# Autodesk Inventor assembly: Сборка крышка
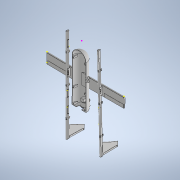
[picture p0: Inventor's stored thumbnail of the model, 180x180]
Saved by Autodesk Inventor 2022.1 (Build 261234000, 234)
## iProperties
Created: 2021-12-25
Part Number: Сборка крышка
Document SubType Name: Assembly
Designer: Grigori
Author: Grigori
## Documents named in this file (19)
- C:\Users\Grigo\Desktop\Дрон\Сборка\Сборка крышка.iam
- C:\Users\Grigo\Desktop\Дрон\Сборка\Корпус1.ipt
- C:\Users\Grigo\Desktop\Дрон\Сборка\Impeller.ipt
- C:\Users\Grigo\Desktop\Дрон\Сборка\Крышка на мотор.ipt
- C:\Users\Grigo\Desktop\Дрон\Сборка\Держатель крыла.ipt
- C:\Users\Grigo\Desktop\Дрон\Сборка\полукрыло.ipt
- C:\Users\Grigo\Desktop\Дрон\Сборка\Продольный фюзеляж.ipt
- C:\Users\Grigo\Desktop\Дрон\Сборка\2207 motor.ipt
- C:\Users\Grigo\Desktop\Дрон\Сборка\esc 80A.ipt
- C:\Users\Grigo\Desktop\Дрон\Сборка\Крышка на ESC.ipt
- C:\Users\Grigo\Desktop\Дрон\Сборка\полукрыло_MIR.ipt
- C:\Users\Grigo\Desktop\Дрон\Сборка\Продольный фюзеляж_MIR.ipt
- C:\Users\Grigo\Desktop\Дрон\Сборка\2207 motor_MIR.ipt
- C:\Users\Grigo\Desktop\Дрон\Сборка\Крышка на ESC_MIR.ipt
- C:\Users\Grigo\Desktop\Дрон\Сборка\esc 80A_MIR.ipt
- C:\Users\Grigo\Documents\Inventor\Content Center Files\R2022\ru-RU\AS 1427(01)\AS 1427 - M3 x 8(3).ipt
- C:\Users\Grigo\Documents\Inventor\Content Center Files\R2022\ru-RU\Rivet JB_T 10582-2006\Rivet JB_T 10582-2006-10 X 25.ipt
- C:\Users\Grigo\Documents\Inventor\Content Center Files\R2022\ru-RU\AS 1427(05)\AS 1427 - M2,5 x 10(5) II.ipt
- C:\Users\Grigo\Documents\Inventor\Content Center Files\R2022\ru-RU\AS 1427(01)\AS 1427 - M3 x 5(3).ipt
## Components (85 placed, 18 different names)
1. Корпус1:1 — С поворотом:1, Совмещение:2, С поворотом:3, С поворотом:4, Жесткий:1, Совмещение:5, Совмещение:25, Совмещение:26, Совмещение:27, Совмещение:28, Совмещение:45
2. Impeller:1 — С поворотом:1, С поворотом:2, Совмещение:45
3. Крышка на мотор:1 — С поворотом:2, Совмещение:2, С поворотом:3, Совмещение:46, Совмещение:47, Совмещение:48, Совмещение:49
4. Держатель крыла:1 — Жесткий:1, Совмещение:3
5. Держатель крыла:2 — С поворотом:4, Совмещение:4
6. полукрыло:1 — Совмещение:3, Совмещение:4, Совмещение:5, Совмещение:6, Совмещение:7, Совмещение:50, Совмещение:51, Совмещение:52
7. Продольный фюзеляж:1 — Совмещение:6, Совмещение:7, Совмещение:8, Совмещение:9, Совмещение:10, Совмещение:11, Совмещение:12, Совмещение:13, Совмещение:14, Совмещение:15, Совмещение:16, Совмещение:17, Совмещение:18, Совмещение:19, Совмещение:20, Совмещение:21, Совмещение:22, Совмещение:23, Совмещение:24, С поворотом:5, С поворотом:6, С поворотом:7, С поворотом:8, С поворотом:9, С поворотом:10, С поворотом:11, С поворотом:12, С поворотом:13, С поворотом:14, С поворотом:15, С поворотом:16
8. 2207 motor:1 — Совмещение:8, Совмещение:11
9. 2207 motor:2 — Совмещение:9, Совмещение:12
10. 2207 motor:3 — Совмещение:10, Совмещение:13
11. esc 80A:1 — Совмещение:14
12. esc 80A:2 — Совмещение:15
13. esc 80A:3 — Совмещение:16
14. Крышка на ESC:1 — Совмещение:22, Совмещение:23, Совмещение:24, С поворотом:37, С поворотом:38, С поворотом:39, С поворотом:40
15. Крышка на ESC:2 — Совмещение:17, Совмещение:18, С поворотом:33, С поворотом:34, С поворотом:35, С поворотом:36
16. Крышка на ESC:3 — Совмещение:19, Совмещение:20, Совмещение:21, С поворотом:29, С поворотом:30, С поворотом:31, С поворотом:32
17. полукрыло_MIR:1 — Совмещение:29, Совмещение:30, Совмещение:53, Совмещение:54, Совмещение:55
18. Продольный фюзеляж_MIR:1 — Совмещение:29, Совмещение:30, Совмещение:31, Совмещение:32, Совмещение:33, Совмещение:34, Совмещение:35, Совмещение:36, Совмещение:37, Совмещение:38, Совмещение:39, Совмещение:40, Совмещение:41, Совмещение:42, Совмещение:43, Совмещение:44, С поворотом:17, С поворотом:18, С поворотом:19, С поворотом:20, С поворотом:21, С поворотом:22, С поворотом:23, С поворотом:24, С поворотом:25, С поворотом:26, С поворотом:27, С поворотом:28
19. 2207 motor_MIR:1 — Совмещение:31, Совмещение:32
20. 2207 motor_MIR:2 — Совмещение:33, Совмещение:34
21. 2207 motor_MIR:3 — Совмещение:35, Совмещение:36
22. Крышка на ESC_MIR:1 — Совмещение:37, Совмещение:38, Совмещение:39, С поворотом:41, С поворотом:42, С поворотом:43, С поворотом:44
23. Крышка на ESC_MIR:2 — Совмещение:40, Совмещение:41, С поворотом:45, С поворотом:46, С поворотом:47, С поворотом:48
24. Крышка на ESC_MIR:3 — Совмещение:42, Совмещение:43, Совмещение:44, С поворотом:49, С поворотом:50, С поворотом:51, С поворотом:52
25. esc 80A_MIR:1
26. esc 80A_MIR:2
27. esc 80A_MIR:3
28. AS 1427 - метрическая M3 x 8:1 — Совмещение:46
29. AS 1427 - метрическая M3 x 8:2 — Совмещение:48
30. AS 1427 - метрическая M3 x 8:3 — Совмещение:47
31. AS 1427 - метрическая M3 x 8:4 — Совмещение:49
32. Rivet JB/T 10582-2006 10 X 25:1 — Совмещение:52
33. Rivet JB/T 10582-2006 10 X 25:2 — Совмещение:51
34. Rivet JB/T 10582-2006 10 X 25:3 — Совмещение:50
35. Rivet JB/T 10582-2006 10 X 25:4 — Совмещение:55
36. Rivet JB/T 10582-2006 10 X 25:5 — Совмещение:54
37. Rivet JB/T 10582-2006 10 X 25:6 — Совмещение:53
38. AS 1427 H - метрическая M2,5 x 10:1 — С поворотом:5
39. AS 1427 H - метрическая M2,5 x 10:2 — С поворотом:8
40. AS 1427 H - метрическая M2,5 x 10:3 — С поворотом:7
41. AS 1427 H - метрическая M2,5 x 10:4 — С поворотом:6
42. AS 1427 H - метрическая M2,5 x 10:5 — С поворотом:9
43. AS 1427 H - метрическая M2,5 x 10:6 — С поворотом:10
44. AS 1427 H - метрическая M2,5 x 10:7 — С поворотом:11
45. AS 1427 H - метрическая M2,5 x 10:8 — С поворотом:12
46. AS 1427 H - метрическая M2,5 x 10:9 — С поворотом:16
47. AS 1427 H - метрическая M2,5 x 10:10 — С поворотом:15
48. AS 1427 H - метрическая M2,5 x 10:11 — С поворотом:13
49. AS 1427 H - метрическая M2,5 x 10:12 — С поворотом:14
50. AS 1427 H - метрическая M2,5 x 10:13 — С поворотом:19
51. AS 1427 H - метрическая M2,5 x 10:14 — С поворотом:17
52. AS 1427 H - метрическая M2,5 x 10:15 — С поворотом:18
53. AS 1427 H - метрическая M2,5 x 10:16 — С поворотом:20
54. AS 1427 H - метрическая M2,5 x 10:17 — С поворотом:22
55. AS 1427 H - метрическая M2,5 x 10:18 — С поворотом:21
56. AS 1427 H - метрическая M2,5 x 10:19 — С поворотом:23
57. AS 1427 H - метрическая M2,5 x 10:20 — С поворотом:24
58. AS 1427 H - метрическая M2,5 x 10:21 — С поворотом:27
59. AS 1427 H - метрическая M2,5 x 10:22 — С поворотом:25
60. AS 1427 H - метрическая M2,5 x 10:23 — С поворотом:26
61. AS 1427 H - метрическая M2,5 x 10:24 — С поворотом:28
62. AS 1427 - метрическая M3 x 5:1 — С поворотом:29
63. AS 1427 - метрическая M3 x 5:2 — С поворотом:30
64. AS 1427 - метрическая M3 x 5:3 — С поворотом:31
65. AS 1427 - метрическая M3 x 5:4 — С поворотом:32
66. AS 1427 - метрическая M3 x 5:5 — С поворотом:34
67. AS 1427 - метрическая M3 x 5:6 — С поворотом:33
68. AS 1427 - метрическая M3 x 5:7 — С поворотом:35
69. AS 1427 - метрическая M3 x 5:8 — С поворотом:36
70. AS 1427 - метрическая M3 x 5:9 — С поворотом:38
71. AS 1427 - метрическая M3 x 5:10 — С поворотом:37
72. AS 1427 - метрическая M3 x 5:11 — С поворотом:39
73. AS 1427 - метрическая M3 x 5:12 — С поворотом:40
74. AS 1427 - метрическая M3 x 5:13 — С поворотом:41
75. AS 1427 - метрическая M3 x 5:14 — С поворотом:42
76. AS 1427 - метрическая M3 x 5:15 — С поворотом:44
77. AS 1427 - метрическая M3 x 5:16 — С поворотом:43
78. AS 1427 - метрическая M3 x 5:17 — С поворотом:45
79. AS 1427 - метрическая M3 x 5:18 — С поворотом:46
80. AS 1427 - метрическая M3 x 5:19 — С поворотом:48
81. AS 1427 - метрическая M3 x 5:20 — С поворотом:47
82. AS 1427 - метрическая M3 x 5:21 — С поворотом:49
83. AS 1427 - метрическая M3 x 5:22 — С поворотом:50
84. AS 1427 - метрическая M3 x 5:23 — С поворотом:52
85. AS 1427 - метрическая M3 x 5:24 — С поворотом:51
## Relationships (108: Mate 54, RevoluteJoint 52, WeldJoint 1, Symmetry 1)
- С поворотом:1 [RevoluteJoint]: Корпус1:1 ↔ Impeller:1
- С поворотом:2 [RevoluteJoint]: Impeller:1 ↔ Крышка на мотор:1
- Совмещение:2 [Mate]: Корпус1:1 ↔ Крышка на мотор:1
- С поворотом:3 [RevoluteJoint]: Корпус1:1 ↔ Крышка на мотор:1
- С поворотом:4 [RevoluteJoint]: Корпус1:1 ↔ Держатель крыла:2
- Жесткий:1 [WeldJoint]: Корпус1:1 ↔ Держатель крыла:1
- Совмещение:3 [Mate]: Держатель крыла:1 ↔ полукрыло:1
- Совмещение:4 [Mate]: Держатель крыла:2 ↔ полукрыло:1
- Совмещение:5 [Mate]: Корпус1:1 ↔ полукрыло:1
- Совмещение:6 [Mate]: полукрыло:1 ↔ Продольный фюзеляж:1
- Совмещение:7 [Mate]: полукрыло:1 ↔ Продольный фюзеляж:1
- Совмещение:8 [Mate]: Продольный фюзеляж:1 ↔ 2207 motor:1
- Совмещение:9 [Mate]: Продольный фюзеляж:1 ↔ 2207 motor:2
- Совмещение:10 [Mate]: Продольный фюзеляж:1 ↔ 2207 motor:3
- Совмещение:11 [Mate]: Продольный фюзеляж:1 ↔ 2207 motor:1
- Совмещение:12 [Mate]: Продольный фюзеляж:1 ↔ 2207 motor:2
- Совмещение:13 [Mate]: Продольный фюзеляж:1 ↔ 2207 motor:3
- Совмещение:14 [Mate]: Продольный фюзеляж:1 ↔ esc 80A:1
- Совмещение:15 [Mate]: Продольный фюзеляж:1 ↔ esc 80A:2
- Совмещение:16 [Mate]: Продольный фюзеляж:1 ↔ esc 80A:3
- Совмещение:17 [Mate]: Продольный фюзеляж:1 ↔ Крышка на ESC:2
- Совмещение:18 [Mate]: Продольный фюзеляж:1 ↔ Крышка на ESC:2
- Совмещение:19 [Mate]: Продольный фюзеляж:1 ↔ Крышка на ESC:3
- Совмещение:20 [Mate]: Продольный фюзеляж:1 ↔ Крышка на ESC:3
- Совмещение:21 [Mate]: Продольный фюзеляж:1 ↔ Крышка на ESC:3
- Совмещение:22 [Mate]: Продольный фюзеляж:1 ↔ Крышка на ESC:1
- Совмещение:23 [Mate]: Продольный фюзеляж:1 ↔ Крышка на ESC:1
- Совмещение:24 [Mate]: Продольный фюзеляж:1 ↔ Крышка на ESC:1
- Совмещение:25 [Mate]: Корпус1:1
- Совмещение:26 [Mate]: Корпус1:1
- Совмещение:27 [Mate]: Корпус1:1
- Совмещение:28 [Mate]: Корпус1:1
- Симметрия:1 [Symmetry]
- Совмещение:29 [Mate]: полукрыло_MIR:1 ↔ Продольный фюзеляж_MIR:1
- Совмещение:30 [Mate]: полукрыло_MIR:1 ↔ Продольный фюзеляж_MIR:1
- Совмещение:31 [Mate]: Продольный фюзеляж_MIR:1 ↔ 2207 motor_MIR:1
- Совмещение:32 [Mate]: Продольный фюзеляж_MIR:1 ↔ 2207 motor_MIR:1
- Совмещение:33 [Mate]: Продольный фюзеляж_MIR:1 ↔ 2207 motor_MIR:2
- Совмещение:34 [Mate]: Продольный фюзеляж_MIR:1 ↔ 2207 motor_MIR:2
- Совмещение:35 [Mate]: Продольный фюзеляж_MIR:1 ↔ 2207 motor_MIR:3
- Совмещение:36 [Mate]: Продольный фюзеляж_MIR:1 ↔ 2207 motor_MIR:3
- Совмещение:37 [Mate]: Продольный фюзеляж_MIR:1 ↔ Крышка на ESC_MIR:1
- Совмещение:38 [Mate]: Продольный фюзеляж_MIR:1 ↔ Крышка на ESC_MIR:1
- Совмещение:39 [Mate]: Продольный фюзеляж_MIR:1 ↔ Крышка на ESC_MIR:1
- Совмещение:40 [Mate]: Продольный фюзеляж_MIR:1 ↔ Крышка на ESC_MIR:2
- Совмещение:41 [Mate]: Продольный фюзеляж_MIR:1 ↔ Крышка на ESC_MIR:2
- Совмещение:42 [Mate]: Продольный фюзеляж_MIR:1 ↔ Крышка на ESC_MIR:3
- Совмещение:43 [Mate]: Продольный фюзеляж_MIR:1 ↔ Крышка на ESC_MIR:3
- Совмещение:44 [Mate]: Продольный фюзеляж_MIR:1 ↔ Крышка на ESC_MIR:3
- Совмещение:45 [Mate]: Корпус1:1 ↔ Impeller:1
- Совмещение:46 [Mate]: Крышка на мотор:1 ↔ AS 1427 - метрическая M3 x 8:1
- Совмещение:47 [Mate]: Крышка на мотор:1 ↔ AS 1427 - метрическая M3 x 8:3
- Совмещение:48 [Mate]: Крышка на мотор:1 ↔ AS 1427 - метрическая M3 x 8:2
- Совмещение:49 [Mate]: Крышка на мотор:1 ↔ AS 1427 - метрическая M3 x 8:4
- Совмещение:50 [Mate]: полукрыло:1 ↔ Rivet JB/T 10582-2006 10 X 25:3
- Совмещение:51 [Mate]: полукрыло:1 ↔ Rivet JB/T 10582-2006 10 X 25:2
- Совмещение:52 [Mate]: полукрыло:1 ↔ Rivet JB/T 10582-2006 10 X 25:1
- Совмещение:53 [Mate]: полукрыло_MIR:1 ↔ Rivet JB/T 10582-2006 10 X 25:6
- Совмещение:54 [Mate]: полукрыло_MIR:1 ↔ Rivet JB/T 10582-2006 10 X 25:5
- Совмещение:55 [Mate]: полукрыло_MIR:1 ↔ Rivet JB/T 10582-2006 10 X 25:4
- С поворотом:5 [RevoluteJoint]: Продольный фюзеляж:1 ↔ AS 1427 H - метрическая M2,5 x 10:1
- С поворотом:6 [RevoluteJoint]: Продольный фюзеляж:1 ↔ AS 1427 H - метрическая M2,5 x 10:4
- С поворотом:7 [RevoluteJoint]: Продольный фюзеляж:1 ↔ AS 1427 H - метрическая M2,5 x 10:3
- С поворотом:8 [RevoluteJoint]: Продольный фюзеляж:1 ↔ AS 1427 H - метрическая M2,5 x 10:2
- С поворотом:9 [RevoluteJoint]: Продольный фюзеляж:1 ↔ AS 1427 H - метрическая M2,5 x 10:5
- С поворотом:10 [RevoluteJoint]: Продольный фюзеляж:1 ↔ AS 1427 H - метрическая M2,5 x 10:6
- С поворотом:11 [RevoluteJoint]: Продольный фюзеляж:1 ↔ AS 1427 H - метрическая M2,5 x 10:7
- С поворотом:12 [RevoluteJoint]: Продольный фюзеляж:1 ↔ AS 1427 H - метрическая M2,5 x 10:8
- С поворотом:13 [RevoluteJoint]: Продольный фюзеляж:1 ↔ AS 1427 H - метрическая M2,5 x 10:11
- С поворотом:14 [RevoluteJoint]: Продольный фюзеляж:1 ↔ AS 1427 H - метрическая M2,5 x 10:12
- С поворотом:15 [RevoluteJoint]: Продольный фюзеляж:1 ↔ AS 1427 H - метрическая M2,5 x 10:10
- С поворотом:16 [RevoluteJoint]: Продольный фюзеляж:1 ↔ AS 1427 H - метрическая M2,5 x 10:9
- С поворотом:17 [RevoluteJoint]: Продольный фюзеляж_MIR:1 ↔ AS 1427 H - метрическая M2,5 x 10:14
- С поворотом:18 [RevoluteJoint]: Продольный фюзеляж_MIR:1 ↔ AS 1427 H - метрическая M2,5 x 10:15
- С поворотом:19 [RevoluteJoint]: Продольный фюзеляж_MIR:1 ↔ AS 1427 H - метрическая M2,5 x 10:13
- С поворотом:20 [RevoluteJoint]: Продольный фюзеляж_MIR:1 ↔ AS 1427 H - метрическая M2,5 x 10:16
- С поворотом:21 [RevoluteJoint]: Продольный фюзеляж_MIR:1 ↔ AS 1427 H - метрическая M2,5 x 10:18
- С поворотом:22 [RevoluteJoint]: Продольный фюзеляж_MIR:1 ↔ AS 1427 H - метрическая M2,5 x 10:17
- С поворотом:23 [RevoluteJoint]: Продольный фюзеляж_MIR:1 ↔ AS 1427 H - метрическая M2,5 x 10:19
- С поворотом:24 [RevoluteJoint]: Продольный фюзеляж_MIR:1 ↔ AS 1427 H - метрическая M2,5 x 10:20
- С поворотом:25 [RevoluteJoint]: Продольный фюзеляж_MIR:1 ↔ AS 1427 H - метрическая M2,5 x 10:22
- С поворотом:26 [RevoluteJoint]: Продольный фюзеляж_MIR:1 ↔ AS 1427 H - метрическая M2,5 x 10:23
- С поворотом:27 [RevoluteJoint]: Продольный фюзеляж_MIR:1 ↔ AS 1427 H - метрическая M2,5 x 10:21
- С поворотом:28 [RevoluteJoint]: Продольный фюзеляж_MIR:1 ↔ AS 1427 H - метрическая M2,5 x 10:24
- С поворотом:29 [RevoluteJoint]: Крышка на ESC:3 ↔ AS 1427 - метрическая M3 x 5:1
- С поворотом:30 [RevoluteJoint]: Крышка на ESC:3 ↔ AS 1427 - метрическая M3 x 5:2
- С поворотом:31 [RevoluteJoint]: Крышка на ESC:3 ↔ AS 1427 - метрическая M3 x 5:3
- С поворотом:32 [RevoluteJoint]: Крышка на ESC:3 ↔ AS 1427 - метрическая M3 x 5:4
- С поворотом:33 [RevoluteJoint]: Крышка на ESC:2 ↔ AS 1427 - метрическая M3 x 5:6
- С поворотом:34 [RevoluteJoint]: Крышка на ESC:2 ↔ AS 1427 - метрическая M3 x 5:5
- С поворотом:35 [RevoluteJoint]: Крышка на ESC:2 ↔ AS 1427 - метрическая M3 x 5:7
- С поворотом:36 [RevoluteJoint]: Крышка на ESC:2 ↔ AS 1427 - метрическая M3 x 5:8
- С поворотом:37 [RevoluteJoint]: Крышка на ESC:1 ↔ AS 1427 - метрическая M3 x 5:10
- С поворотом:38 [RevoluteJoint]: Крышка на ESC:1 ↔ AS 1427 - метрическая M3 x 5:9
- С поворотом:39 [RevoluteJoint]: Крышка на ESC:1 ↔ AS 1427 - метрическая M3 x 5:11
- С поворотом:40 [RevoluteJoint]: Крышка на ESC:1 ↔ AS 1427 - метрическая M3 x 5:12
- С поворотом:41 [RevoluteJoint]: Крышка на ESC_MIR:1 ↔ AS 1427 - метрическая M3 x 5:13
- С поворотом:42 [RevoluteJoint]: Крышка на ESC_MIR:1 ↔ AS 1427 - метрическая M3 x 5:14
- С поворотом:43 [RevoluteJoint]: Крышка на ESC_MIR:1 ↔ AS 1427 - метрическая M3 x 5:16
- С поворотом:44 [RevoluteJoint]: Крышка на ESC_MIR:1 ↔ AS 1427 - метрическая M3 x 5:15
- С поворотом:45 [RevoluteJoint]: Крышка на ESC_MIR:2 ↔ AS 1427 - метрическая M3 x 5:17
- С поворотом:46 [RevoluteJoint]: Крышка на ESC_MIR:2 ↔ AS 1427 - метрическая M3 x 5:18
- С поворотом:47 [RevoluteJoint]: Крышка на ESC_MIR:2 ↔ AS 1427 - метрическая M3 x 5:20
- С поворотом:48 [RevoluteJoint]: Крышка на ESC_MIR:2 ↔ AS 1427 - метрическая M3 x 5:19
- С поворотом:49 [RevoluteJoint]: Крышка на ESC_MIR:3 ↔ AS 1427 - метрическая M3 x 5:21
- С поворотом:50 [RevoluteJoint]: Крышка на ESC_MIR:3 ↔ AS 1427 - метрическая M3 x 5:22
- С поворотом:51 [RevoluteJoint]: Крышка на ESC_MIR:3 ↔ AS 1427 - метрическая M3 x 5:24
- С поворотом:52 [RevoluteJoint]: Крышка на ESC_MIR:3 ↔ AS 1427 - метрическая M3 x 5:23
